# Autodesk Inventor assembly: SPE3V1 Freno
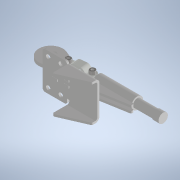
[picture p0: Inventor's stored thumbnail of the model, 180x180]
Saved by Autodesk Inventor 2021.2 (Build 252289000, 289)
## iProperties
Created: 2026-06-23
Part Number: SPE3V1 Freno
Document SubType Name: Assembly
Designer: nelso
Author: nelso
## Documents named in this file (8)
- C:\Users\nelso\Desktop\Soporte-Paciente-Espinografia\Workspace\SPE3V1 Freno.iam
- C:\Users\nelso\Desktop\Soporte-Paciente-Espinografia\Workspace\base_cuerpo_chapa.ipt
- C:\Users\nelso\Desktop\Soporte-Paciente-Espinografia\Workspace\cuerpo_chapa.ipt
- C:\Users\nelso\Desktop\Soporte-Paciente-Espinografia\Workspace\Part4.ipt
- C:\Users\nelso\Desktop\Soporte-Paciente-Espinografia\Workspace\palanca2.ipt
- C:\Users\nelso\Desktop\Soporte-Paciente-Espinografia\Workspace\Viela GH-304-305-CM.ipt
- C:\Users\nelso\Desktop\Soporte-Paciente-Espinografia\Workspace\vastago.ipt
- C:\Users\nelso\Desktop\Soporte-Paciente-Espinografia\Workspace\DIN912-M5X0.8L16P.ipt
## Components (10 placed, 7 different names)
1. base_cuerpo_chapa:1 — Mate:5, Flush:2, Mate:11, Mate:13, Mate:35, Mate:46, Mate:58
2. cuerpo_chapa:1 — Mate:13, Flush:3, Mate:46, Flush:5
3. cuerpo_chapa:2 — Mate:11, Flush:4, Tangent:1, Mate:58
4. palanca2:1 — Mate:34, Mate:38, Mate:61, Mate:62, Mate:65
5. Viela GH-304-305-CM:1 — Mate:59, Mate:60, Mate:61, Mate:63, Mate:64
6. Viela GH-304-305-CM:2 — Mate:65, Mate:66, Mate:67
7. vastago:1 — Mate:41, Mate:57, Flush:6, Mate:68
8. Part4:1 — Mate:33, Mate:40, Tangent:1, Flush:5, Mate:57, Flush:6
9. DIN912-M5X0.8L16P:1 — Mate:59, Mate:60, Mate:62, Mate:66
10. DIN912-M5X0.8L16P:2 — Mate:63, Mate:64, Mate:67, Mate:68
## Relationships (28: Mate 22, Flush 5, Tangent 1)
- Mate:5: base_cuerpo_chapa:1
- Flush:2: base_cuerpo_chapa:1
- Mate:11: base_cuerpo_chapa:1 ↔ cuerpo_chapa:2
- Mate:13: base_cuerpo_chapa:1 ↔ cuerpo_chapa:1
- Mate:33: Part4:1
- Mate:34: palanca2:1
- Flush:3 (4 mm): cuerpo_chapa:1
- Mate:35: base_cuerpo_chapa:1
- Flush:4 (-4 mm): cuerpo_chapa:2
- Mate:38: palanca2:1
- Mate:40: Part4:1
- Tangent:1: cuerpo_chapa:2 ↔ Part4:1
- Mate:41: vastago:1
- Mate:46: base_cuerpo_chapa:1 ↔ cuerpo_chapa:1
- Flush:5: cuerpo_chapa:1 ↔ Part4:1
- Mate:57: vastago:1 ↔ Part4:1
- Flush:6 (-18 mm): vastago:1 ↔ Part4:1
- Mate:58: base_cuerpo_chapa:1 ↔ cuerpo_chapa:2
- Mate:59: Viela GH-304-305-CM:1 ↔ DIN912-M5X0.8L16P:1
- Mate:60: Viela GH-304-305-CM:1 ↔ DIN912-M5X0.8L16P:1
- Mate:61: palanca2:1 ↔ Viela GH-304-305-CM:1
- Mate:62: palanca2:1 ↔ DIN912-M5X0.8L16P:1
- Mate:63: Viela GH-304-305-CM:1 ↔ DIN912-M5X0.8L16P:2
- Mate:64: Viela GH-304-305-CM:1 ↔ DIN912-M5X0.8L16P:2
- Mate:65: palanca2:1 ↔ Viela GH-304-305-CM:2
- Mate:66: Viela GH-304-305-CM:2 ↔ DIN912-M5X0.8L16P:1
- Mate:67: Viela GH-304-305-CM:2 ↔ DIN912-M5X0.8L16P:2
- Mate:68: vastago:1 ↔ DIN912-M5X0.8L16P:2
